# Autodesk Inventor assembly: Pulley Shaft
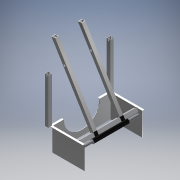
[picture p0: Inventor's stored thumbnail of the model, 180x180]
Saved by Autodesk Inventor 2017 (Build 210142000, 142)
## iProperties
Created: 2020-02-20
Part Number: Pulley Shaft
Document SubType Name: Assembly
Designer: S346553810
Author: S346553810
## Documents named in this file (14)
- \\ad.ocdsb.ca\studenthome\0\S346553810\1.Robotics\1086091_FRC_Season_2020_-_Infinite_Recharge_64c12036a2ea9777_1582146647\FullRobotRefactor\Intake\Pulley Shaft.iam
- \\ad.ocdsb.ca\studenthome\0\S346553810\1.Robotics\1086091_FRC_Season_2020_-_Infinite_Recharge_64c12036a2ea9777_1582146647\FullRobotRefactor\Intake\Intake Drop.ipt
- \\ad.ocdsb.ca\studenthome\0\S346553810\1.Robotics\1086091_FRC_Season_2020_-_Infinite_Recharge_64c12036a2ea9777_1582146647\FullRobotRefactor\Intake\Roller cylinder.ipt
- \\ad.ocdsb.ca\studenthome\0\S346553810\1.Robotics\1086091_FRC_Season_2020_-_Infinite_Recharge_64c12036a2ea9777_1582146647\FullRobotRefactor\Intake\Roller Mount Piece.ipt
- \\ad.ocdsb.ca\studenthome\0\S346553810\1.Robotics\1086091_FRC_Season_2020_-_Infinite_Recharge_64c12036a2ea9777_1582146647\FullRobotRefactor\Intake\TexturedRoller.ipt
- P:\1.Robotics\1086091_FRC_Season_2020_-_Infinite_Recharge_64c12036a2ea9777_1582146647\FullRobotRefactor\SubFrame\1in sq tub - 4.ipt
- P:\1.Robotics\1086091_FRC_Season_2020_-_Infinite_Recharge_64c12036a2ea9777_1582146647\FullRobotRefactor\SubFrame\Kipp K0617.ipt
- P:\1.Robotics\1086091_FRC_Season_2020_-_Infinite_Recharge_64c12036a2ea9777_1582146647\FullRobotRefactor\SubFrame\1in sq tub - 6-5.ipt
- \\ad.ocdsb.ca\studenthome\0\S346553810\1.Robotics\1086091_FRC_Season_2020_-_Infinite_Recharge_64c12036a2ea9777_1582146647\FullRobotRefactor\Intake\conveyer frame.ipt
- \\ad.ocdsb.ca\studenthome\0\S346553810\1.Robotics\1086091_FRC_Season_2020_-_Infinite_Recharge_64c12036a2ea9777_1582146647\FullRobotRefactor\Intake\Convery frame2.ipt
- \\ad.ocdsb.ca\studenthome\0\S346553810\1.Robotics\1086091_FRC_Season_2020_-_Infinite_Recharge_64c12036a2ea9777_1582146647\FullRobotRefactor\Intake\42T Wide Timing Pulley.iam
- P:\1.Robotics\1086091_FRC_Season_2020_-_Infinite_Recharge_64c12036a2ea9777_1582146647\FullRobotRefactor\Intake\RampMount.ipt
- \\ad.ocdsb.ca\studenthome\0\S346553810\1.Robotics\1086091_FRC_Season_2020_-_Infinite_Recharge_64c12036a2ea9777_1582146647\FullRobotRefactor\Intake\VersaPlanetary_v1_Single_Stage_10_1_with_BAG.ipt
- P:\1.Robotics\1086091_FRC_Season_2020_-_Infinite_Recharge_64c12036a2ea9777_1582146647\FullRobotRefactor\Intake\Part3.ipt
## Components (19 placed, 13 different names)
1. Intake Drop:1 — Mate:1, Mate:2, Angle:1, Mate:3, Mate:4, Mate:6, Mate:18, Mate:19, Flush:13, Flush:14, Mate:20, Mate:21
2. Roller cylinder:1 — Mate:5, Mate:6, Mate:7
3. Roller Mount Piece:1 — Mate:1, Mate:2, Angle:1, Flush:1, Mate:5, Mate:8, Mate:9, Flush:2, Flush:3
4. Roller Mount Piece:2 — Mate:3, Mate:4, Flush:1, Flush:4, Flush:5, Mate:10
5. TexturedRoller:1 — Mate:7, Mate:8
6. 1in sq tub - 4:5 — Mate:9, Flush:2, Flush:3, Flush:7, Mate:11, Mate:25
7. 1in sq tub - 4:6 — Flush:4, Flush:5, Mate:10, Flush:6, Mate:12, Mate:13, Flush:9, Flush:15
8. Kipp K0617:6 — Mate:12, Mate:13, Mate:14, Flush:8, Mate:22
9. 1in sq tub - 6-5:1 — Mate:14, Flush:8, Flush:9, Mate:23
10. Kipp K0617:7 — Flush:6, Flush:7, Mate:11, Mate:24, Flush:16
11. Convery frame2:2 — Flush:14, Mate:20, Mate:21
12. Convery frame2:3 — Mate:18, Mate:19, Flush:13, Flush:17, Flush:18
13. conveyer frame:3 — Mate:22, Flush:15, Mate:23, Mate:26, Flush:19, Angle:2
14. conveyer frame:4 — Mate:24, Flush:16, Mate:25, Mate:30, Flush:20, Flush:21
15. RampMount:1 — Flush:17, Flush:18
16. 42T Wide Timing Pulley:1 [sub-assembly] — Mate:27, Mate:28, Mate:30
17. 42T Wide Timing Pulley:2 [sub-assembly] — Mate:28, Mate:29
18. VersaPlanetary_v1_Single_Stage_10_1_with_BAG:1 — Mate:26, Flush:19, Angle:2, Mate:27, Mate:29
19. Part3:1 — Flush:20, Flush:21
## Relationships (47: Mate 27, Flush 18, Angle 2)
- Mate:1: Intake Drop:1 ↔ Roller Mount Piece:1
- Mate:2: Intake Drop:1 ↔ Roller Mount Piece:1
- Angle:1 (58.666 deg): Intake Drop:1 ↔ Roller Mount Piece:1
- Mate:3: Intake Drop:1 ↔ Roller Mount Piece:2
- Mate:4: Intake Drop:1 ↔ Roller Mount Piece:2
- Flush:1: Roller Mount Piece:1 ↔ Roller Mount Piece:2
- Mate:5: Roller cylinder:1 ↔ Roller Mount Piece:1
- Mate:6: Intake Drop:1 ↔ Roller cylinder:1
- Mate:7: Roller cylinder:1 ↔ TexturedRoller:1
- Mate:8 (76.2 mm): Roller Mount Piece:1 ↔ TexturedRoller:1
- Mate:9: Roller Mount Piece:1 ↔ 1in sq tub - 4:5
- Flush:2: Roller Mount Piece:1 ↔ 1in sq tub - 4:5
- Flush:3: Roller Mount Piece:1 ↔ 1in sq tub - 4:5
- Flush:4: Roller Mount Piece:2 ↔ 1in sq tub - 4:6
- Flush:5: Roller Mount Piece:2 ↔ 1in sq tub - 4:6
- Mate:10: Roller Mount Piece:2 ↔ 1in sq tub - 4:6
- Flush:6: 1in sq tub - 4:6 ↔ Kipp K0617:7
- Flush:7: 1in sq tub - 4:5 ↔ Kipp K0617:7
- Mate:11: 1in sq tub - 4:5 ↔ Kipp K0617:7
- Mate:12: 1in sq tub - 4:6 ↔ Kipp K0617:6
- Mate:13: 1in sq tub - 4:6 ↔ Kipp K0617:6
- Mate:14: Kipp K0617:6 ↔ 1in sq tub - 6-5:1
- Flush:8: Kipp K0617:6 ↔ 1in sq tub - 6-5:1
- Flush:9: 1in sq tub - 4:6 ↔ 1in sq tub - 6-5:1
- Mate:18: Intake Drop:1 ↔ Convery frame2:3
- Mate:19: Intake Drop:1 ↔ Convery frame2:3
- Flush:13: Intake Drop:1 ↔ Convery frame2:3
- Flush:14: Intake Drop:1 ↔ Convery frame2:2
- Mate:20: Intake Drop:1 ↔ Convery frame2:2
- Mate:21: Intake Drop:1 ↔ Convery frame2:2
- Mate:22: Kipp K0617:6 ↔ conveyer frame:3
- Flush:15: 1in sq tub - 4:6 ↔ conveyer frame:3
- Mate:23: 1in sq tub - 6-5:1 ↔ conveyer frame:3
- Mate:24: Kipp K0617:7 ↔ conveyer frame:4
- Flush:16: Kipp K0617:7 ↔ conveyer frame:4
- Mate:25: 1in sq tub - 4:5 ↔ conveyer frame:4
- Flush:17: Convery frame2:3 ↔ RampMount:1
- Flush:18: Convery frame2:3 ↔ RampMount:1
- Mate:26: conveyer frame:3 ↔ VersaPlanetary_v1_Single_Stage_10_1_with_BAG:1
- Flush:19: conveyer frame:3 ↔ VersaPlanetary_v1_Single_Stage_10_1_with_BAG:1
- Angle:2 (90 deg): conveyer frame:3 ↔ VersaPlanetary_v1_Single_Stage_10_1_with_BAG:1
- Mate:27 (122.3518 mm): 42T Wide Timing Pulley:1 ↔ VersaPlanetary_v1_Single_Stage_10_1_with_BAG:1
- Mate:28: 42T Wide Timing Pulley:1 ↔ 42T Wide Timing Pulley:2
- Mate:29: 42T Wide Timing Pulley:2 ↔ VersaPlanetary_v1_Single_Stage_10_1_with_BAG:1
- Mate:30: conveyer frame:4 ↔ 42T Wide Timing Pulley:1
- Flush:20: conveyer frame:4 ↔ Part3:1
- Flush:21: conveyer frame:4 ↔ Part3:1
